# Autodesk Inventor assembly: MDL-BDC
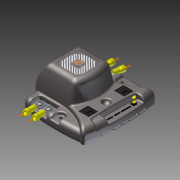
[picture p0: Inventor's stored thumbnail of the model, 180x180]
Saved by Autodesk Inventor 2011 (Build 150239000, 239)
## iProperties
Category: Control System
Company: Autodesk Inc.
Created: 2008-12-09
Part Number: MDL-BDC
Document SubType Name: Assembly
Designer: Autodesk Inc.
Catalog Web Link: http://www.luminarymicro.com/products/mdl_bdc.html
Vendor: Luminary Micro
Description: Motor Controller
Author: Autodesk Inc.
## Documents named in this file (6)
- \\lmss\STUDENTS\Robotics\2012\Inventor\vkop\All-Control-System\MotorController_LuminaryMicro_MDL-BDC.iam
- \\lmss\STUDENTS\Robotics\2012\Inventor\vkop\All-Control-System\Jaguar main enclosure.ipt
- \\lmss\STUDENTS\Robotics\2012\Inventor\vkop\All-Control-System\ANSI B18.6.3 - 8-36 UNF - 0.25(7).ipt
- \\lmss\STUDENTS\Robotics\2012\Inventor\vkop\All-Control-System\IFI - 4(16).ipt
- \\lmss\STUDENTS\Robotics\2012\Inventor\vkop\All-Electrical\RingTerminal_Tyco_35149.ipt
- \\lmss\STUDENTS\Robotics\2012\Inventor\vkop\All-Control-System\MotorController_LuminaryMicro_MDL-BDC\AIP\Cable and Harness\MotorController_LuminaryMicro_MDL-BDC.Harness1.iam
## Components (14 placed, 5 different names)
1. Jaguar main enclosure:1 — Mate:2, Mate:3, Mate:4, Mate:5
2. RingTerminal_Tyco_35149:1 — Insert:3, Mate:12, Mate:14
3. RingTerminal_Tyco_35149:2 — Insert:4, Mate:13, Mate:16
4. RingTerminal_Tyco_35149:3 — Insert:5, Mate:9, Mate:10
5. RingTerminal_Tyco_35149:4 — Insert:6, Mate:6, Mate:7
6. Harness1 [sub-assembly]
7. Cross Recessed Pan Head Machine Screw - Type II - Inch No. 8 - 36 - 1/4:1 — Mate:2, Insert:1
8. Square Test Washer (Metric) (IFI) 4:1 — Insert:1, Mate:3, Angle:1, Insert:3
9. Cross Recessed Pan Head Machine Screw - Type II - Inch No. 8 - 36 - 1/4:5
10. Square Test Washer (Metric) (IFI) 4:2 — Insert:4
11. Cross Recessed Pan Head Machine Screw - Type II - Inch No. 8 - 36 - 1/4:6 — Insert:2
12. Square Test Washer (Metric) (IFI) 4:3 — Angle:2, Insert:2, Insert:5, Mate:5
13. Cross Recessed Pan Head Machine Screw - Type II - Inch No. 8 - 36 - 1/4:7
14. Square Test Washer (Metric) (IFI) 4:4 — Insert:6, Mate:4
## Component patterns: (2 elements, first: Cross Recessed Pan Head Machine Screw - Type II - Inch No. 8 - 36 - 1/4:1 + Square Test Washer (Metric) (IFI) 4:1), (2 elements, first: Cross Recessed Pan Head Machine Screw - Type II - Inch No. 8 - 36 - 1/4:6 + Square Test Washer (Metric) (IFI) 4:3)
## Relationships (24: Mate 16, Insert 6, Angle 2)
- Mate:2: Jaguar main enclosure:1 ↔ Cross Recessed Pan Head Machine Screw - Type II - Inch No. 8 - 36 - 1/4:1
- Insert:1: Cross Recessed Pan Head Machine Screw - Type II - Inch No. 8 - 36 - 1/4:1 ↔ Square Test Washer (Metric) (IFI) 4:1
- Mate:3 (1.27 mm): Jaguar main enclosure:1 ↔ Square Test Washer (Metric) (IFI) 4:1
- Angle:1 (0 deg): Square Test Washer (Metric) (IFI) 4:1
- Angle:2 (0 deg): Square Test Washer (Metric) (IFI) 4:3
- Insert:2: Cross Recessed Pan Head Machine Screw - Type II - Inch No. 8 - 36 - 1/4:6 ↔ Square Test Washer (Metric) (IFI) 4:3
- Insert:3: RingTerminal_Tyco_35149:1 ↔ Square Test Washer (Metric) (IFI) 4:1
- Insert:4: RingTerminal_Tyco_35149:2 ↔ Square Test Washer (Metric) (IFI) 4:2
- Insert:5: RingTerminal_Tyco_35149:3 ↔ Square Test Washer (Metric) (IFI) 4:3
- Insert:6: RingTerminal_Tyco_35149:4 ↔ Square Test Washer (Metric) (IFI) 4:4
- Mate:4: Jaguar main enclosure:1 ↔ Square Test Washer (Metric) (IFI) 4:4
- Mate:5: Jaguar main enclosure:1 ↔ Square Test Washer (Metric) (IFI) 4:3
- Mate:6: RingTerminal_Tyco_35149:4
- Mate:7: RingTerminal_Tyco_35149:4
- Mate:8
- Mate:9: RingTerminal_Tyco_35149:3
- Mate:10: RingTerminal_Tyco_35149:3
- Mate:11
- Mate:12: RingTerminal_Tyco_35149:1
- Mate:13: RingTerminal_Tyco_35149:2
- Mate:14: RingTerminal_Tyco_35149:1
- Mate:15
- Mate:16: RingTerminal_Tyco_35149:2
- Mate:17
